# Autodesk Inventor assembly: DepthSensor
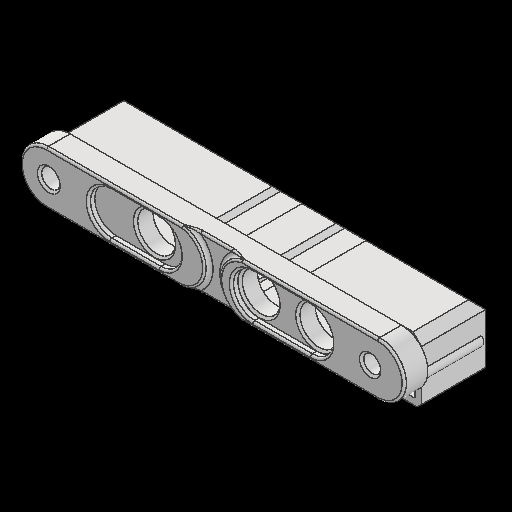
[picture p0: Inventor's stored thumbnail of the model, 512x512]
Saved by Autodesk Inventor 2025.2 (Build 292293000, 293)
## iProperties
Created: 2026-02-04
Part Number: DepthSensor
Document SubType Name: Assembly
Designer: valer
Author: valer
## Documents named in this file (3)
- C:\Users\valer\Desktop\str1ker\cad\DepthSensor.iam
- C:\Users\valer\Desktop\str1ker\cad\DepthCameraHousing.ipt
- C:\Users\valer\Desktop\str1ker\cad\external\DepthSensor\PrimeSenseCarmine1.09-Cover.ipt
## Components (2 placed, 2 different names)
1. DepthCameraHousing:1 — Mate:1, Flush:1
2. PrimeSenseCarmine1.09-Cover:1 — Mate:1, Flush:1
## Relationships (2: Mate 1, Flush 1)
- Mate:1: DepthCameraHousing:1 ↔ PrimeSenseCarmine1.09-Cover:1
- Flush:1: DepthCameraHousing:1 ↔ PrimeSenseCarmine1.09-Cover:1
